# Autodesk Inventor assembly: SQUICK_full
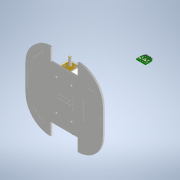
[picture p0: Inventor's stored thumbnail of the model, 180x180]
Saved by Autodesk Inventor 2020.3 (Build 243373000, 373)
## iProperties
Created: 2021-03-17
Part Number: SQUICK_full
Document SubType Name: Assembly
Designer: patry
Author: patry
## Documents named in this file (5)
- C:\Users\patry\Desktop\MM Squick\squick_inventor\Workspace\SQUICK_full.iam
- C:\Users\patry\Desktop\MM Squick\squick_inventor\Workspace\Board_base\board_base.ipt
- C:\Users\patry\Desktop\MM Squick\squick_inventor\Workspace\Motor with brace\micro-metal-gearmotor-extended-with-1089-extended-bracket.ipt
- C:\Users\patry\Desktop\MM Squick\squick_inventor\Workspace\Encoders\magnetic-encoder-pair-kit-for-micro-metal-gearmotors-hpcb-compatible\magnetic-encoder-pair-kit-for-micro-metal-gearmotors-hpcb-compatible-enc0.ipt
- C:\Users\patry\Desktop\MM Squick\squick_inventor\Workspace\Encoders\magnetic-encoder-pair-kit-for-micro-metal-gearmotors-hpcb-compatible\magnetic-encoder-pair-kit-for-micro-metal-gearmotors-hpcb-compatible-w1r0.ipt
## Components (7 placed, 4 different names)
1. board_base:1 — Zestawiające:1, Zestawiające:2, Równoległe:1, Równoległe:2, Zestawiające:3, Zestawiające:4, Kątowe:1
2. micro-metal-gearmotor-extended-with-1089-extended-bracket:1 — Zestawiające:1, Równoległe:1, Zestawiające:4, Zestawiające:5, Zestawiające:7, Zestawiające:8
3. micro-metal-gearmotor-extended-with-1089-extended-bracket:2 — Zestawiające:2, Równoległe:2, Zestawiające:3, Zestawiające:6
4. magnetic-encoder-pair-kit-for-micro-metal-gearmotors-hpcb-compatible-enc0:1 — Zestawiające:7, Zestawiające:8, Zestawiające:9, Kątowe:1
5. magnetic-encoder-pair-kit-for-micro-metal-gearmotors-hpcb-compatible-w1r0:1 — Zestawiające:5, Zestawiające:9
6. magnetic-encoder-pair-kit-for-micro-metal-gearmotors-hpcb-compatible-enc0:2
7. magnetic-encoder-pair-kit-for-micro-metal-gearmotors-hpcb-compatible-w1r0:2 — Zestawiające:6
## Relationships (12: Mate 9, Flush 2, Angle 1)
- Zestawiające:1 [Mate] (4 mm): board_base:1 ↔ micro-metal-gearmotor-extended-with-1089-extended-bracket:1
- Zestawiające:2 [Mate]: board_base:1 ↔ micro-metal-gearmotor-extended-with-1089-extended-bracket:2
- Równoległe:1 [Flush] (-0.5 mm): board_base:1 ↔ micro-metal-gearmotor-extended-with-1089-extended-bracket:1
- Równoległe:2 [Flush] (-0.5 mm): board_base:1 ↔ micro-metal-gearmotor-extended-with-1089-extended-bracket:2
- Zestawiające:3 [Mate]: board_base:1 ↔ micro-metal-gearmotor-extended-with-1089-extended-bracket:2
- Zestawiające:4 [Mate]: board_base:1 ↔ micro-metal-gearmotor-extended-with-1089-extended-bracket:1
- Zestawiające:5 [Mate]: micro-metal-gearmotor-extended-with-1089-extended-bracket:1 ↔ magnetic-encoder-pair-kit-for-micro-metal-gearmotors-hpcb-compatible-w1r0:1
- Zestawiające:6 [Mate]: micro-metal-gearmotor-extended-with-1089-extended-bracket:2 ↔ magnetic-encoder-pair-kit-for-micro-metal-gearmotors-hpcb-compatible-w1r0:2
- Zestawiające:7 [Mate]: micro-metal-gearmotor-extended-with-1089-extended-bracket:1 ↔ magnetic-encoder-pair-kit-for-micro-metal-gearmotors-hpcb-compatible-enc0:1
- Zestawiające:8 [Mate]: micro-metal-gearmotor-extended-with-1089-extended-bracket:1 ↔ magnetic-encoder-pair-kit-for-micro-metal-gearmotors-hpcb-compatible-enc0:1
- Zestawiające:9 [Mate] (0.5 mm): magnetic-encoder-pair-kit-for-micro-metal-gearmotors-hpcb-compatible-enc0:1 ↔ magnetic-encoder-pair-kit-for-micro-metal-gearmotors-hpcb-compatible-w1r0:1
- Kątowe:1 [Angle] (180 deg): board_base:1 ↔ magnetic-encoder-pair-kit-for-micro-metal-gearmotors-hpcb-compatible-enc0:1
